# Autodesk Inventor assembly: maniac
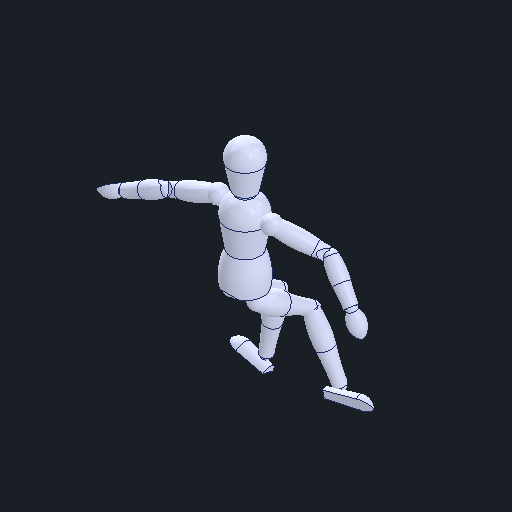
[picture p0: Inventor's stored thumbnail of the model, 512x512]
Saved by Autodesk Inventor 2025.3 (Build 293356000, 356)
## iProperties
Created: 2026-08-12
Part Number: maniac
Document SubType Name: Assembly
Designer: VianaCC
Author: VianaCC
## Documents named in this file (12)
- C:\Users\vianacc\Documents\GitHub\utv_startup\products\utv\ergonomics\cad\reference\maniac.iam
- C:\Users\vianacc\Documents\suporte_capacete\Arm\Arm.ipt
- C:\Users\vianacc\Documents\suporte_capacete\Body\Body.ipt
- C:\Users\vianacc\Documents\suporte_capacete\Femur\Femur.ipt
- C:\Users\vianacc\Documents\suporte_capacete\Foot\Foot.ipt
- C:\Users\vianacc\Documents\suporte_capacete\Forearm\Forearm.ipt
- C:\Users\vianacc\Documents\suporte_capacete\Hand\Hand.ipt
- C:\Users\vianacc\Documents\suporte_capacete\Head\Head.ipt
- C:\Users\vianacc\Documents\suporte_capacete\Hip\Hip.ipt
- C:\Users\vianacc\Documents\suporte_capacete\Pelvis\Pelvis.ipt
- C:\Users\vianacc\Documents\suporte_capacete\Sura\Sura.ipt
- C:\Users\vianacc\Documents\suporte_capacete\Waist\Waist.ipt
## Components (18 placed, 11 different names)
1. Head:1 — Mate:1, Flush:1, Angle:1
2. Body:1 — Mate:1, Mate:2, Mate:5, Mate:13, Flush:1, Angle:1, Mate:19, Angle:21
3. Pelvis:1 — Mate:6, Mate:7, Mate:17, Mate:19, Angle:21, Angle:22, Angle:23, Angle:24, Angle:25
4. Waist:1 — Mate:5, Mate:6
5. Arm:1 — Mate:2, Mate:3
6. Forearm:1 — Mate:3, Mate:4
7. Hand:1 — Mate:4
8. Arm:2 — Mate:13
9. Forearm:2
10. Hand:2
11. Femur:1 — Mate:9, Mate:18, Angle:22, Angle:23
12. Foot:1 — Mate:10
13. Hip:1 — Mate:7, Mate:18
14. Sura:1 — Mate:9, Mate:10
15. Femur:2 — Angle:24, Angle:25
16. Foot:2
17. Hip:2 — Mate:17
18. Sura:2
## Relationships (25: Mate 18, Angle 6, Flush 1)
- Mate:1: Head:1 ↔ Body:1
- Mate:2: Body:1 ↔ Arm:1
- Mate:3: Arm:1 ↔ Forearm:1
- Mate:4: Forearm:1 ↔ Hand:1
- Mate:5: Body:1 ↔ Waist:1
- Mate:6: Pelvis:1 ↔ Waist:1
- Mate:7: Pelvis:1 ↔ Hip:1
- Mate:9: Femur:1 ↔ Sura:1
- Mate:10: Foot:1 ↔ Sura:1
- [Mate]: Arm:2 ↔ Forearm:2
- [Mate]: Forearm:2 ↔ Hand:2
- Mate:13: Body:1 ↔ Arm:2
- [Mate]: Femur:2 ↔ Hip:2
- [Mate]: Femur:2 ↔ Sura:2
- [Mate]: Foot:2 ↔ Sura:2
- Mate:17: Pelvis:1 ↔ Hip:2
- Mate:18: Femur:1 ↔ Hip:1
- Flush:1: Head:1 ↔ Body:1
- Angle:1 (0 deg): Head:1 ↔ Body:1
- Mate:19: Body:1 ↔ Pelvis:1
- Angle:21 (180 deg): Body:1 ↔ Pelvis:1
- Angle:22 (5 deg): Pelvis:1 ↔ Femur:1
- Angle:23 (60 deg): Pelvis:1 ↔ Femur:1
- Angle:24 (-60 deg): Pelvis:1 ↔ Femur:2
- Angle:25 (5 deg): Pelvis:1 ↔ Femur:2
## Named parameters: d10_d2 = 0 mm, d11_d3 = 0 mm, d13_d7 = 0 mm, d14_d8 = 0 mm, d15_d9 = 0 mm, headbody = 0 deg, bodypelvis = 180 deg
